# Autodesk Inventor assembly: Assembly2
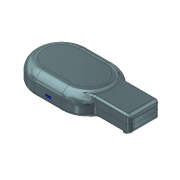
[picture p0: Inventor's stored thumbnail of the model, 180x180]
Saved by Autodesk Inventor 2022.1 (Build 261234020, 234B)
## iProperties
Created: 2022-10-03
Part Number: Assembly2
Document SubType Name: Assembly
Designer: HP
Author: HP
## Documents named in this file (13)
- C:\Users\HP\OneDrive\Documentos\Inventor\BIODEÑO\Assembly2.iam
- C:\Users\HP\OneDrive\Documentos\Inventor\BIODEÑO\Carcasa 1.ipt
- C:\Users\HP\OneDrive\Documentos\Inventor\BIODEÑO\HX711.ipt
- C:\Users\HP\OneDrive\Documentos\Inventor\BIODEÑO\ESP-WROOM32.ipt
- C:\Users\HP\OneDrive\Documentos\Inventor\BIODEÑO\Carcasa 2.ipt
- C:\Users\HP\OneDrive\Documentos\Inventor\BIODEÑO\1S 4056 BMS USB C Module 01b.ipt
- C:\Users\HP\OneDrive\Documentos\Inventor\BIODEÑO\interruptor patilla recortada.ipt
- C:\Users\HP\OneDrive\Documentos\Inventor\BIODEÑO\Bateria LiPo 3.7V 1000mA 503450 v23.ipt
- C:\Users\HP\OneDrive\Documentos\Inventor\BIODEÑO\Cella_car.ipt
- C:\Users\HP\OneDrive\Documentos\Inventor\BIODEÑO\LED 5mm.ipt
- C:\Users\HP\OneDrive\Documentos\Inventor\BIODEÑO\MAX17043.ipt
- C:\Users\HP\OneDrive\Documentos\Inventor\BIODEÑO\MINIPROTOBOARD.ipt
- C:\Users\HP\OneDrive\Documentos\Inventor\BIODEÑO\BARRA.ipt
## Components (12 placed, 12 different names)
1. Carcasa 1:1 — Mate:1, Mate:2, Mate:3, Mate:4, Mate:5, Flush:1, Mate:15
2. Carcasa 2:1 — Mate:1, Mate:2, Mate:3, Mate:6, Mate:7, Flush:2, Mate:8, Mate:9, Mate:11, Mate:12, Mate:13, Mate:14, Mate:16, Mate:17, Mate:18
3. 1S 4056 BMS USB C Module 01b:1 — Mate:6, Mate:7, Flush:2
4. ESP-WROOM32:1
5. HX711:1 — Mate:12
6. interruptor patilla recortada:1 — Mate:8, Mate:9
7. Bateria LiPo 3.7V 1000mA 503450 v23:1 — Mate:17
8. Cella_car:1 — Mate:15, Mate:16
9. LED 5mm:2 — Mate:11
10. MAX17043:1 — Mate:14
11. MINIPROTOBOARD:1 — Mate:13
12. BARRA:1 — Mate:18
## Relationships (19: Mate 17, Flush 2)
- Mate:1: Carcasa 1:1 ↔ Carcasa 2:1
- Mate:2: Carcasa 1:1 ↔ Carcasa 2:1
- Mate:3: Carcasa 1:1 ↔ Carcasa 2:1
- Mate:4: Carcasa 1:1
- Mate:5: Carcasa 1:1
- Flush:1: Carcasa 1:1
- Mate:6: Carcasa 2:1 ↔ 1S 4056 BMS USB C Module 01b:1
- Mate:7: Carcasa 2:1 ↔ 1S 4056 BMS USB C Module 01b:1
- Flush:2: Carcasa 2:1 ↔ 1S 4056 BMS USB C Module 01b:1
- Mate:8: Carcasa 2:1 ↔ interruptor patilla recortada:1
- Mate:9: Carcasa 2:1 ↔ interruptor patilla recortada:1
- Mate:11: Carcasa 2:1 ↔ LED 5mm:2
- Mate:12: Carcasa 2:1 ↔ HX711:1
- Mate:13: Carcasa 2:1 ↔ MINIPROTOBOARD:1
- Mate:14: Carcasa 2:1 ↔ MAX17043:1
- Mate:15: Carcasa 1:1 ↔ Cella_car:1
- Mate:16: Carcasa 2:1 ↔ Cella_car:1
- Mate:17: Carcasa 2:1 ↔ Bateria LiPo 3.7V 1000mA 503450 v23:1
- Mate:18: Carcasa 2:1 ↔ BARRA:1
